# Autodesk Inventor assembly: CD+Airfoils
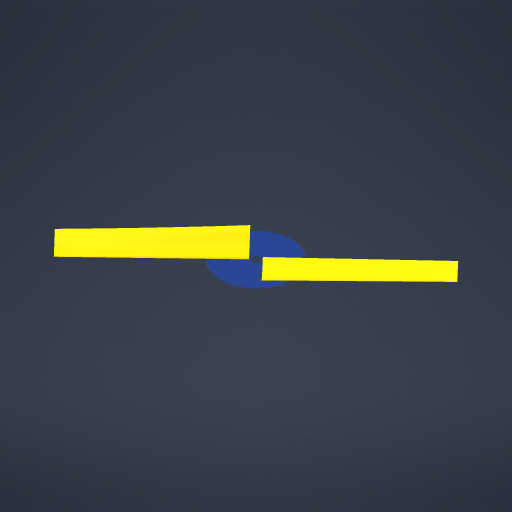
[picture p0: Inventor's stored thumbnail of the model, 512x512]
Saved by Autodesk Inventor 2024.1 (Build 281209000, 209)
## iProperties
Created: 2024-11-17
Part Number: CD+Airfoils
Document SubType Name: Assembly
Designer: Designer
Author: Designer
## Documents named in this file (3)
- C:\Users\Designer\Desktop\optics\CD+Airfoils.iam
- C:\Users\Designer\Desktop\optics\CD.ipt
- C:\Users\Designer\Desktop\optics\BladeV1.ipt
## Components (3 placed, 2 different names)
1. CD:1 — Mate:5, Flush:1
2. BladeV1:1 — Mate:1, Mate:2
3. BladeV1:2 — Mate:3, Mate:4
## Relationships (6: Mate 5, Flush 1)
- Mate:1: BladeV1:1
- Mate:2: BladeV1:1
- Mate:3: BladeV1:2
- Mate:4: BladeV1:2
- Mate:5: CD:1
- Flush:1: CD:1
